# Autodesk Inventor assembly: Z-Axis Transmission Assembly Front
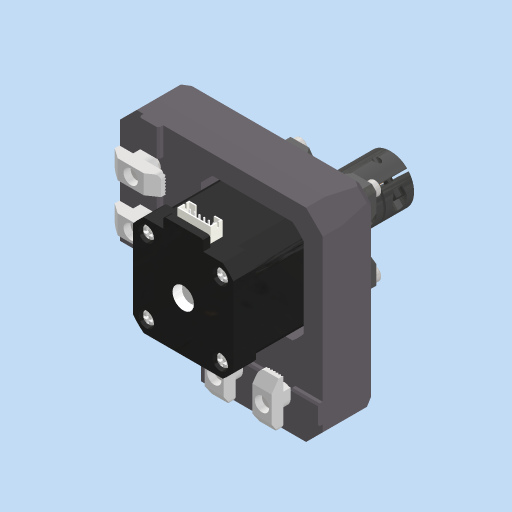
[picture p0: Inventor's stored thumbnail of the model, 512x512]
Saved by Autodesk Inventor 2023.2 (Build 272271000, 271)
## iProperties
Created: 2023-11-23
Part Number: Z-Axis Transmission Assembly Front
Document SubType Name: Assembly
Designer: Nils Bade
Author: Nils Bade
## Documents named in this file (9)
- C:\Users\nilsb\Documents\Inventor\Projektarbeit-Bade\RatRig_Bade\Z-Axis Transmission Assembly Front.iam
- C:\Users\nilsb\Documents\Inventor\Projektarbeit-Bade\RatRig_modified\Leadscrew Motorcage Front for 4040.ipt
- C:\Users\nilsb\Documents\Inventor\Projektarbeit-Bade\RatRig_Standards\Nema 17 Stepper Motor - 48mm - 1.8degree_step, 76oz-in v1.ipt
- C:\Users\nilsb\Documents\Inventor\Projektarbeit-Bade\Schrauben\Cap Head Screw M6x20 v2.ipt
- C:\Users\nilsb\Documents\Inventor\Projektarbeit-Bade\RatRig_modified\T-NUT - DropIn 4040 SERIES - M6.ipt
- C:\Users\nilsb\Documents\Inventor\Projektarbeit-Bade\RatRig_Standards\pillow_block v2.ipt
- C:\Users\nilsb\Documents\Inventor\Projektarbeit-Bade\Schrauben\Cap Head Screw M3x18 v2.ipt
- C:\Users\nilsb\Documents\Inventor\Projektarbeit-Bade\RatRig_Standards\Thrust Bearing F8-16M v1.ipt
- C:\Users\nilsb\Documents\Inventor\Projektarbeit-Bade\RatRig_Standards\Coupler - Rigid Type - Black 25x20mm - 5mm to 8mm v2.iam
## Components (17 placed, 8 different names)
1. Leadscrew Motorcage Front for 4040:1 — Passend:1, Winkel:1, Passend:2, Passend:4, Passend:5, Passend:14, Passend:15, Passend:16, Passend:17, Passend:18, Passend:19, Passend:20, Passend:21, Passend:26, Passend:27, Passend:28, Passend:29, Winkel:2, Winkel:3, Winkel:4, Winkel:5
2. Nema 17 Stepper Motor - 48mm - 1.8degree_step, 76oz-in v1:1 — Passend:1, Winkel:1, Passend:2, Passend:3, Passend:30, Passend:32
3. Cap Head Screw M6x20 v2:1 — Passend:14, Passend:21, Passend:23
4. Cap Head Screw M6x20 v2:2 — Passend:15, Passend:20, Passend:22
5. Cap Head Screw M6x20 v2:3 — Passend:16, Passend:19, Passend:24
6. Cap Head Screw M6x20 v2:4 — Passend:17, Passend:18, Passend:25
7. T-NUT - DROP IN TYPE FOR 40 SERIES - M6:1 — Passend:23, Passend:29, Winkel:3
8. T-NUT - DROP IN TYPE FOR 40 SERIES - M6:2 — Passend:22, Passend:28, Winkel:2
9. T-NUT - DROP IN TYPE FOR 40 SERIES - M6:3 — Passend:24, Passend:27, Winkel:4
10. T-NUT - DROP IN TYPE FOR 40 SERIES - M6:4 — Passend:25, Passend:26, Winkel:5
11. pillow_block v2:1 — Passend:3, Passend:4, Passend:5, Passend:6, Passend:7, Passend:8, Passend:9, Passend:10, Passend:11, Passend:12, Passend:13, Passend:31
12. Cap Head Screw M3x18 v2:1 — Passend:7, Passend:11
13. Cap Head Screw M3x18 v2:2 — Passend:8, Passend:10
14. Cap Head Screw M3x18 v2:3 — Passend:9, Passend:12
15. Cap Head Screw M3x18 v2:4 — Passend:6, Passend:13
16. Thrust Bearing F8-16M v1:1 — Passend:30, Passend:31, Passend:33
17. Coupler - Rigid Type - Black 25x20mm - 5mm to 8mm v2:1 [sub-assembly] — Passend:32, Passend:33
## Relationships (38: Mate 33, Angle 5)
- Passend:1 [Mate]: Leadscrew Motorcage Front for 4040:1 ↔ Nema 17 Stepper Motor - 48mm - 1.8degree_step, 76oz-in v1:1
- Winkel:1 [Angle] (0 deg): Leadscrew Motorcage Front for 4040:1 ↔ Nema 17 Stepper Motor - 48mm - 1.8degree_step, 76oz-in v1:1
- Passend:2 [Mate]: Leadscrew Motorcage Front for 4040:1 ↔ Nema 17 Stepper Motor - 48mm - 1.8degree_step, 76oz-in v1:1
- Passend:3 [Mate]: Nema 17 Stepper Motor - 48mm - 1.8degree_step, 76oz-in v1:1 ↔ pillow_block v2:1
- Passend:4 [Mate]: Leadscrew Motorcage Front for 4040:1 ↔ pillow_block v2:1
- Passend:5 [Mate]: Leadscrew Motorcage Front for 4040:1 ↔ pillow_block v2:1
- Passend:6 [Mate]: pillow_block v2:1 ↔ Cap Head Screw M3x18 v2:4
- Passend:7 [Mate]: pillow_block v2:1 ↔ Cap Head Screw M3x18 v2:1
- Passend:8 [Mate]: pillow_block v2:1 ↔ Cap Head Screw M3x18 v2:2
- Passend:9 [Mate]: pillow_block v2:1 ↔ Cap Head Screw M3x18 v2:3
- Passend:10 [Mate]: pillow_block v2:1 ↔ Cap Head Screw M3x18 v2:2
- Passend:11 [Mate]: pillow_block v2:1 ↔ Cap Head Screw M3x18 v2:1
- Passend:12 [Mate]: pillow_block v2:1 ↔ Cap Head Screw M3x18 v2:3
- Passend:13 [Mate]: pillow_block v2:1 ↔ Cap Head Screw M3x18 v2:4
- Passend:14 [Mate]: Leadscrew Motorcage Front for 4040:1 ↔ Cap Head Screw M6x20 v2:1
- Passend:15 [Mate]: Leadscrew Motorcage Front for 4040:1 ↔ Cap Head Screw M6x20 v2:2
- Passend:16 [Mate]: Leadscrew Motorcage Front for 4040:1 ↔ Cap Head Screw M6x20 v2:3
- Passend:17 [Mate]: Leadscrew Motorcage Front for 4040:1 ↔ Cap Head Screw M6x20 v2:4
- Passend:18 [Mate]: Leadscrew Motorcage Front for 4040:1 ↔ Cap Head Screw M6x20 v2:4
- Passend:19 [Mate]: Leadscrew Motorcage Front for 4040:1 ↔ Cap Head Screw M6x20 v2:3
- Passend:20 [Mate]: Leadscrew Motorcage Front for 4040:1 ↔ Cap Head Screw M6x20 v2:2
- Passend:21 [Mate]: Leadscrew Motorcage Front for 4040:1 ↔ Cap Head Screw M6x20 v2:1
- Passend:22 [Mate]: Cap Head Screw M6x20 v2:2 ↔ T-NUT - DROP IN TYPE FOR 40 SERIES - M6:2
- Passend:23 [Mate]: Cap Head Screw M6x20 v2:1 ↔ T-NUT - DROP IN TYPE FOR 40 SERIES - M6:1
- Passend:24 [Mate]: Cap Head Screw M6x20 v2:3 ↔ T-NUT - DROP IN TYPE FOR 40 SERIES - M6:3
- Passend:25 [Mate]: Cap Head Screw M6x20 v2:4 ↔ T-NUT - DROP IN TYPE FOR 40 SERIES - M6:4
- Passend:26 [Mate] (4.5 mm): Leadscrew Motorcage Front for 4040:1 ↔ T-NUT - DROP IN TYPE FOR 40 SERIES - M6:4
- Passend:27 [Mate] (4.5 mm): Leadscrew Motorcage Front for 4040:1 ↔ T-NUT - DROP IN TYPE FOR 40 SERIES - M6:3
- Passend:28 [Mate] (4.5 mm): Leadscrew Motorcage Front for 4040:1 ↔ T-NUT - DROP IN TYPE FOR 40 SERIES - M6:2
- Passend:29 [Mate] (4.5 mm): Leadscrew Motorcage Front for 4040:1 ↔ T-NUT - DROP IN TYPE FOR 40 SERIES - M6:1
- Winkel:2 [Angle] (0 deg): Leadscrew Motorcage Front for 4040:1 ↔ T-NUT - DROP IN TYPE FOR 40 SERIES - M6:2
- Winkel:3 [Angle] (0 deg): Leadscrew Motorcage Front for 4040:1 ↔ T-NUT - DROP IN TYPE FOR 40 SERIES - M6:1
- Winkel:4 [Angle] (0 deg): Leadscrew Motorcage Front for 4040:1 ↔ T-NUT - DROP IN TYPE FOR 40 SERIES - M6:3
- Winkel:5 [Angle] (0 deg): Leadscrew Motorcage Front for 4040:1 ↔ T-NUT - DROP IN TYPE FOR 40 SERIES - M6:4
- Passend:30 [Mate]: Nema 17 Stepper Motor - 48mm - 1.8degree_step, 76oz-in v1:1 ↔ Thrust Bearing F8-16M v1:1
- Passend:31 [Mate]: pillow_block v2:1 ↔ Thrust Bearing F8-16M v1:1
- Passend:32 [Mate]: Nema 17 Stepper Motor - 48mm - 1.8degree_step, 76oz-in v1:1 ↔ Coupler - Rigid Type - Black 25x20mm - 5mm to 8mm v2:1
- Passend:33 [Mate]: Thrust Bearing F8-16M v1:1 ↔ Coupler - Rigid Type - Black 25x20mm - 5mm to 8mm v2:1
